# Autodesk Inventor assembly: populated-keyboard_cherrymx
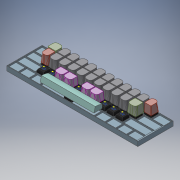
[picture p0: Inventor's stored thumbnail of the model, 180x180]
Saved by Autodesk Inventor 2016 (Build 200138000, 138)
## iProperties
Created: 2016-12-08
Part Number: populated-keyboard_cherrymx
Document SubType Name: Assembly
Designer: Cemra JC
Author: Cemra JC
## Documents named in this file (10)
- J:\The Files\The Software Files\Projects\stenotoppers\cherrymx\base-model\mockup-parts\populated-keyboard_cherrymx.iam
- J:\The Files\The Software Files\Projects\stenotoppers\cherrymx\base-model\mockup-parts\keyboard-mockup_cherrymx.iam
- J:\The Files\The Software Files\Projects\stenotoppers\cherrymx\base-model\mockup-parts\cherry-mx-switch\keyswitch_cherrymx.iam
- J:\The Files\The Software Files\Projects\stenotoppers\cherrymx\base-model\mockup-parts\spacebar-keycap_mockup_cherrymx.ipt
- J:\The Files\The Software Files\Projects\stenotoppers\cherrymx\base-model\base-keycap\standard_cmx.ipt
- J:\The Files\The Software Files\Projects\stenotoppers\cherrymx\base-model\base-keycap.ipt
- J:\The Files\The Software Files\Projects\stenotoppers\cherrymx\base-model\base-keycap\smaller_cmx.ipt
- J:\The Files\The Software Files\Projects\stenotoppers\cherrymx\base-model\base-keycap\larger_cmx.ipt
- J:\The Files\The Software Files\Projects\stenotoppers\cherrymx\base-model\base-keycap\thumb_cmx.ipt
- J:\The Files\The Software Files\Projects\stenotoppers\parameters.xlsx
## Components (30 placed, 9 different names)
1. keyboard-mockup_cherrymx:1 [sub-assembly] — Spacebar Switch Attachment, Rigid:11, Rigid:12, Rigid:13, Rigid:14, Rigid:15, Rigid:16, Rigid:17, Rigid:18
2. Larger Left — Rigid:14
3. Smaller Right — Rigid:18
4. Smaller Left — Rigid:13
5. Larger Right — Rigid:17
6. spacebar-keyswitch [sub-assembly] — Spacebar Switch Attachment, Spacebar Attachment
7. spacebar-keycap_mockup_cherrymx:1 — Spacebar Attachment
8. standard_cmx:1 — Rigid:11
9. standard_cmx:9
10. standard_cmx:10
11. standard_cmx:11
12. standard_cmx:12
13. standard_cmx:13
14. standard_cmx:14
15. standard_cmx:15
16. standard_cmx:16
17. standard_cmx:17
18. standard_cmx:2 — Rigid:12
19. standard_cmx:18
20. standard_cmx:19
21. standard_cmx:20
22. standard_cmx:21
23. standard_cmx:22
24. standard_cmx:23
25. standard_cmx:24
26. standard_cmx:25
27. thumb_cmx:7 — Rigid:15
28. thumb_cmx:26
29. thumb_cmx:8 — Rigid:16
30. thumb_cmx:27
## Component patterns: Top Row (10 elements), Middle Row (9 elements), Thumbs Left (2 elements), Thumbs Right (2 elements)
## Relationships (10: WeldJoint 10)
- Spacebar Switch Attachment [WeldJoint]: keyboard-mockup_cherrymx:1 ↔ spacebar-keyswitch
- Spacebar Attachment [WeldJoint]: spacebar-keyswitch ↔ spacebar-keycap_mockup_cherrymx:1
- Rigid:11 [WeldJoint]: keyboard-mockup_cherrymx:1 ↔ standard_cmx:1
- Rigid:12 [WeldJoint]: keyboard-mockup_cherrymx:1 ↔ standard_cmx:2
- Rigid:13 [WeldJoint]: keyboard-mockup_cherrymx:1 ↔ Smaller Left
- Rigid:14 [WeldJoint]: keyboard-mockup_cherrymx:1 ↔ Larger Left
- Rigid:15 [WeldJoint]: keyboard-mockup_cherrymx:1 ↔ thumb_cmx:7
- Rigid:16 [WeldJoint]: keyboard-mockup_cherrymx:1 ↔ thumb_cmx:8
- Rigid:17 [WeldJoint]: keyboard-mockup_cherrymx:1 ↔ Larger Right
- Rigid:18 [WeldJoint]: keyboard-mockup_cherrymx:1 ↔ Smaller Right
## Named parameters: k_width = 18.1 mm, k_height = 18 mm, k_height_t = 16 mm, k_taper1 = 1.5 mm, k_taper2 = 0.5 mm, k_staper = 1 mm, k_sradius = 4 mm, k_ltaper = 1.5 mm, k_lradius = 6 mm, k_radius = 6 mm, k_wthick = 1.5 mm, k_ribthick = 1.5 mm, k_ribheight = 5 mm, k_poleoff = 2.2625 mm, k_poledia = 5.54 mm, k_cmxw = 1.35 mm, k_cmxl = 4.4 mm, s_bwidth = 15.6 mm, s_poleh = 3.6 mm, s_polebw = 5.5 mm, s_polebl = 7 mm, b_pad = 1 mm, b_tab = 27.15 mm, b_caps = 31.675 mm, b_lshift = 40.725 mm, b_rshift = 49.775 mm, b_ctrl = 22.625 mm, b_space = 117.65 mm, b_width = 286.5 mm, b_height = 77.4 mm, k_taper_thin = 0.5 mm, k_height_low = 16 mm, k_taper_wide = 1.5 mm
